# Autodesk Inventor assembly: EDMPumpRegionAssembly
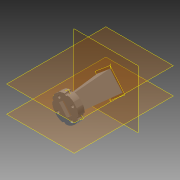
[picture p0: Inventor's stored thumbnail of the model, 180x180]
Saved by Autodesk Inventor 2013 (Build 170138000, 138)
## iProperties
Created: 2014-03-24
Part Number: EDMPumpRegionAssembly
Document SubType Name: Assembly
Designer: jad211
Author: jad211
## Documents named in this file (3)
- C:\CADFiles\EDM New Pumping Region\EDMPumpRegionAssembly.iam
- C:\CADFiles\EDM New Pumping Region\NewHorn.ipt
- C:\CADFiles\EDM New Pumping Region\WG18FLANGECutDown.ipt
## Components (3 placed, 2 different names)
1. NewHorn:1 — Flush:9, Flush:10, Mate:1, Mate:2, Mate:4, Mate:6, Mate:7
2. WG18FLANGECutDown:1 — Flush:10, Mate:1, Mate:2, Mate:3, Mate:5
3. WG18FLANGECutDown:2 — Mate:3, Mate:4, Mate:5, Mate:6
## Relationships (12: Mate 7, Flush 5)
- Flush:6 (17 mm)
- Flush:7 (-17 mm)
- Flush:8 (3 mm)
- Flush:9: NewHorn:1
- Flush:10: NewHorn:1 ↔ WG18FLANGECutDown:1
- Mate:1: NewHorn:1 ↔ WG18FLANGECutDown:1
- Mate:2: NewHorn:1 ↔ WG18FLANGECutDown:1
- Mate:3: WG18FLANGECutDown:1 ↔ WG18FLANGECutDown:2
- Mate:4: NewHorn:1 ↔ WG18FLANGECutDown:2
- Mate:5: WG18FLANGECutDown:1 ↔ WG18FLANGECutDown:2
- Mate:6: NewHorn:1 ↔ WG18FLANGECutDown:2
- Mate:7 (6 mm): NewHorn:1
